# Autodesk Inventor assembly: BandaTrans1
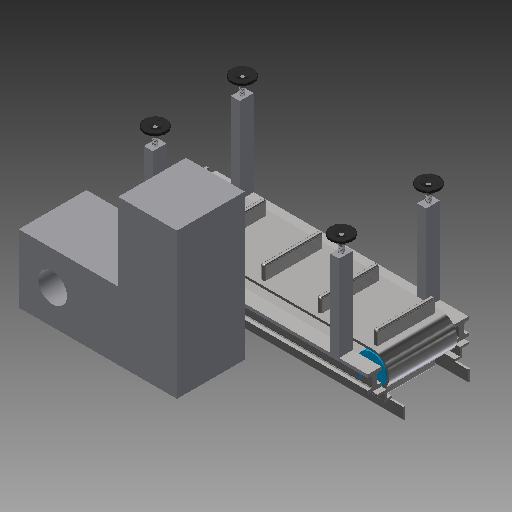
[picture p0: Inventor's stored thumbnail of the model, 512x512]
Saved by Autodesk Inventor 2019 (Build 230136000, 136)
## iProperties
Created: 2019-03-24
Part Number: BandaTrans1
Document SubType Name: Assembly
Designer: felix
Mass: 14687.3 g
Surface Area: 14199.6 cm^2
Volume: 14687.3 cm^3
Density: 1 g/cm^3
Author: felix
## Documents named in this file (8)
- D:\Documents\Inventor\Content Center Files\BandaTrans1.iam
- D:\Documents\Inventor\banda.ipt
- D:\Documents\Inventor\Content Center Files\Rodo.ipt
- D:\Documents\Inventor\Content Center Files\Barra.ipt
- D:\Documents\Inventor\Content Center Files\gancho1.ipt
- D:\Documents\Inventor\Content Center Files\gancho.ipt
- D:\Downloads\Assembly v7\Leveling leg M10 v3.iam
- D:\Documents\Inventor\Content Center Files\stand.ipt
## Components (12 placed, 7 different names)
1. banda:1 — Mate:1, Mate:2, Cylindrical:1, Cylindrical:2, Flush:1, Flush:2
2. Rodo:1 — Cylindrical:1, Flush:1, Rotational:1, Rotational:3
3. Rodo:2 — Cylindrical:2, Flush:2, Rotational:2, Rotational:4
4. Barra:1 — Rotational:1, Rotational:2, Flush:5, Mate:4, Flush:6, Rigid:1, Rigid:3
5. Barra:2 — Rotational:3, Rotational:4, Flush:3, Mate:3, Flush:4, Rigid:2, Rigid:4
6. gancho1:1 — Flush:3, Mate:3, Flush:4
7. gancho:1 — Flush:5, Mate:4, Flush:6
8. Leveling leg M10 v3:2 [sub-assembly] — Rigid:3
9. Leveling leg M10 v3:3 [sub-assembly] — Rigid:2
10. Leveling leg M10 v3:4 [sub-assembly] — Rigid:1
11. Leveling leg M10 v3:5 [sub-assembly] — Rigid:4
12. stand:1 — Flush:7, Mate:5, Mate:6
## Relationships (23: Flush 7, Mate 6, RevoluteJoint 4, WeldJoint 4, CylindricalJoint 2)
- Mate:1: banda:1
- Mate:2: banda:1
- Cylindrical:1: banda:1 ↔ Rodo:1
- Cylindrical:2: banda:1 ↔ Rodo:2
- Flush:1 (2.5 mm): banda:1 ↔ Rodo:1
- Flush:2 (2.5 mm): banda:1 ↔ Rodo:2
- Rotational:1 [RevoluteJoint]: Rodo:1 ↔ Barra:1
- Rotational:2 [RevoluteJoint]: Rodo:2 ↔ Barra:1
- Rotational:3 [RevoluteJoint]: Rodo:1 ↔ Barra:2
- Rotational:4 [RevoluteJoint]: Rodo:2 ↔ Barra:2
- Flush:3: Barra:2 ↔ gancho1:1
- Mate:3: Barra:2 ↔ gancho1:1
- Flush:4: Barra:2 ↔ gancho1:1
- Flush:5: Barra:1 ↔ gancho:1
- Mate:4: Barra:1 ↔ gancho:1
- Flush:6: Barra:1 ↔ gancho:1
- Rigid:1 [WeldJoint]: Barra:1 ↔ Leveling leg M10 v3:4
- Rigid:2 [WeldJoint]: Barra:2 ↔ Leveling leg M10 v3:3
- Rigid:3 [WeldJoint]: Barra:1 ↔ Leveling leg M10 v3:2
- Rigid:4 [WeldJoint]: Barra:2 ↔ Leveling leg M10 v3:5
- Flush:7 (50 mm): stand:1
- Mate:5 (-583 mm): stand:1
- Mate:6 (247 mm): stand:1
